# Autodesk Inventor assembly: CamAssemblyExample
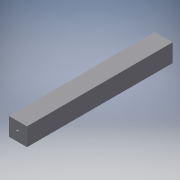
[picture p0: Inventor's stored thumbnail of the model, 180x180]
Saved by Autodesk Inventor 2017 (Build 210142000, 142)
## iProperties
Created: 2016-05-08
Part Number: CamAssemblyExample
Document SubType Name: Assembly
Designer: steele
Author: steele
## Documents named in this file (3)
- C:\snobotics\CAD-Development\robSteele\SnoBotics2016\LinearExample\CamAssemblyExample.iam
- C:\snobotics\CAD-Development\robSteele\SnoBotics2016\LinearExample\LinearExample.ipt
- C:\snobotics\CAD-Development\robSteele\SnoBotics2016\LinearExample\Piston.ipt
## Components (2 placed, 2 different names)
1. LinearExample:1 — Insert:1
2. Piston:1 — Insert:1
## Relationships (1: Insert 1)
- Insert:1: LinearExample:1 ↔ Piston:1
